# Autodesk Inventor assembly: 4mm Dyneema Cable Pulley Bracket
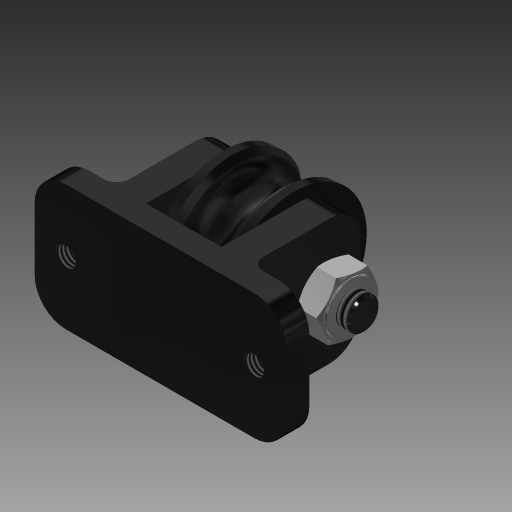
[picture p0: Inventor's stored thumbnail of the model, 512x512]
Saved by Autodesk Inventor 2023 (Build 270158000, 158)
## iProperties
Created: 2023-01-02
Part Number: 4mm Dyneema Cable Pulley Bracket
Document SubType Name: Assembly
Designer: Max Boord
Mass: 60.1854 g
Surface Area: 115.434 cm^2
Volume: 19.7529 cm^3
Density: 3.04692 g/cm^3
Author: Max Boord
## Documents named in this file (9)
- E:\Collaborative Robots\Collaborative Part Library\Elevators\ThriftyBot Elevator Parts\4mm Dyneema Cable Pulley Bracket.iam
- E:\Collaborative Robots\Collaborative Part Library\Elevators\ThriftyBot Elevator Parts\TTB 4mm Dyneema Cable Pulley Bracket (ELEV-PULLEY-001).ipt
- E:\Collaborative Robots\Collaborative Part Library\Elevators\ThriftyBot Elevator Parts\TTB 4mm Dyneema Cable Pulley.ipt
- E:\Collaborative Robots\Collaborative Part Library\Hardware\Fasteners\Machine Screws\1(_FS)4-20 UNCx1.375 Button Head Cap Screw.ipt
- E:\Collaborative Robots\Collaborative Part Library\Hardware\Fasteners\Machine Screws.ipt
- E:\Collaborative Robots\Collaborative Part Library\Hardware\Nuts and Threaded Blocks\Nuts\1(_FS)4(_DQ)-20 Pan Head Nylon locknut.ipt
- E:\Collaborative Robots\Collaborative Part Library\Hardware\Nuts and Threaded Blocks\Nuts.ipt
- E:\Collaborative Robots\Collaborative Part Library\Power Transfer\Bearings and Bushings\Bearings\R188ZZ.ipt
- E:\Collaborative Robots\Collaborative Part Library\Power Transfer\Bearings and Bushings\Bearings.ipt
## Components (6 placed, 5 different names)
1. TTB 4mm Dyneema Cable Pulley Bracket (ELEV-PULLEY-001):1
2. TTB 4mm Dyneema Cable Pulley:1
3. 1(_FS)4-20 UNCx1.375 Button Head Cap Screw:1
4. 1(_FS)4(_DQ)-20 Pan Head Nylon locknut:1
5. R188ZZ:1
6. R188ZZ:2
## Relationships (6: Insert 4, Mate 2)
- [Mate]: TTB 4mm Dyneema Cable Pulley Bracket (ELEV-PULLEY-001):1 ↔ TTB 4mm Dyneema Cable Pulley:1
- [Mate]: TTB 4mm Dyneema Cable Pulley Bracket (ELEV-PULLEY-001):1 ↔ TTB 4mm Dyneema Cable Pulley:1
- [Insert]: TTB 4mm Dyneema Cable Pulley Bracket (ELEV-PULLEY-001):1 ↔ 1(_FS)4(_DQ)-20 Pan Head Nylon locknut:1
- [Insert]: TTB 4mm Dyneema Cable Pulley Bracket (ELEV-PULLEY-001):1 ↔ 1(_FS)4-20 UNCx1.375 Button Head Cap Screw:1
- [Insert]: TTB 4mm Dyneema Cable Pulley:1 ↔ R188ZZ:1
- [Insert]: TTB 4mm Dyneema Cable Pulley:1 ↔ R188ZZ:2
## Named parameters: d651_d378 = 0 mm, d652_d379 = 0 mm, d653_d362_d332 = 0 mm, d654_d363_d333 = 0 mm, d655_d364_d334 = 0 mm, d656_d365_d335 = 0 mm
